# Autodesk Inventor assembly: Wax Seal   b
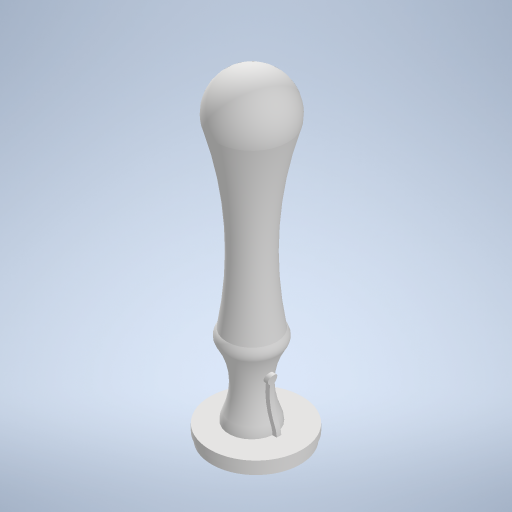
[picture p0: Inventor's stored thumbnail of the model, 512x512]
Saved by Autodesk Inventor 2024 (Build 280153000, 153)
## iProperties
Created: 2023-05-18
Part Number: Wax Seal   b
Document SubType Name: Assembly
Designer: newic
Author: newic
## Documents named in this file (3)
- D:\.My Models\.Inventor\Wax Seal\Wax Seal   b.iam
- D:\.My Models\.Inventor\Wax Seal\Basic seal circle handel a.ipt
- D:\.My Models\.Inventor\Wax Seal\Basic seal circle head    b.ipt
## Components (2 placed, 2 different names)
1. Basic seal circle handel a:1 — Mate:1, Mate:2
2. Basic seal circle head    b:1 — Mate:1, Mate:2
## Relationships (2: Mate 2)
- Mate:1: Basic seal circle handel a:1 ↔ Basic seal circle head    b:1
- Mate:2: Basic seal circle handel a:1 ↔ Basic seal circle head    b:1
